# Autodesk Inventor assembly: Box_Tray_Assembly
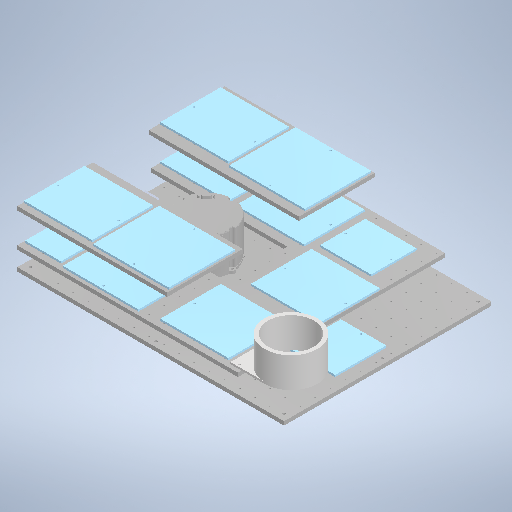
[picture p0: Inventor's stored thumbnail of the model, 512x512]
Saved by Autodesk Inventor 2025.3 (Build 293356000, 356)
## iProperties
Created: 2026-02-04
Part Number: Box_Tray_Assembly
Document SubType Name: Assembly
Designer: m263126
Author: m263126
## Documents named in this file (12)
- C:\Users\m263126\Documents\EW401 Capstone\CAD Files\Box_Tray_Assembly.iam
- C:\Users\m263126\Documents\EW401 Capstone\CAD Files\Box_Body.ipt
- C:\Users\m263126\Documents\EW401 Capstone\CAD Files\box tray_base.ipt
- C:\Users\m263126\Documents\EW401 Capstone\CAD Files\box tray_middle.ipt
- C:\Users\m263126\Documents\EW401 Capstone\CAD Files\box tray_top.ipt
- C:\Users\m263126\Documents\EW401 Capstone\CAD Files\Sensors\TAC-450\TAC-450 IMU.iam
- C:\Users\m263126\Documents\EW401 Capstone\CAD Files\Sensors\VN\vn100_rugged v2.iam
- C:\Users\m263126\Documents\EW401 Capstone\CAD Files\Brackets\4x2_bracket.ipt
- C:\Users\m263126\Documents\EW401 Capstone\CAD Files\Brackets\5x4_bracket.ipt
- C:\Users\m263126\Documents\EW401 Capstone\CAD Files\Brackets\4x4_bracket.ipt
- C:\Users\m263126\Documents\EW401 Capstone\CAD Files\Brackets\3x3_bracket.ipt
- C:\Users\m263126\Documents\EW401 Capstone\CAD Files\Brackets\Battery_holder2.ipt
## Components (19 placed, 11 different names)
1. Box_Body:1 — Mate:3, Mate:4
2. box tray_base:1 — Flush:1, Flush:2, Mate:1, Mate:3, Mate:4, Mate:5, Mate:6, Mate:7, Mate:8, Mate:9, Mate:41, Mate:42, Mate:43
3. box tray_middle:1 — Flush:1, Flush:2, Mate:1, Flush:3, Flush:4, Mate:2, Mate:25, Mate:26, Mate:27, Mate:28, Mate:29, Mate:30, Mate:31, Mate:33, Mate:34, Mate:37, Mate:38, Mate:39, Mate:40, Mate:44, Mate:45, Mate:46, Mate:47, Mate:48, Mate:49
4. box tray_top:1 — Flush:3, Flush:4, Mate:2, Mate:50, Mate:51, Mate:52, Mate:53, Mate:54, Mate:55, Mate:56, Mate:57, Mate:58, Mate:59, Mate:60, Mate:61
5. TAC-450 IMU:1 [sub-assembly] — Mate:5, Mate:6, Mate:7
6. vn100_rugged v2:1 [sub-assembly] — Mate:8, Mate:9
7. 4x4_bracket:2 — Mate:25, Mate:29, Mate:33
8. 4x4_bracket:3 — Mate:26, Mate:30, Mate:34
9. 4x4_bracket:4 — Mate:27
10. 4x4_bracket:5 — Mate:28, Mate:31, Mate:37
11. 5x4_bracket:1 — Mate:38, Mate:39, Mate:40
12. 5x4_bracket:2 — Mate:56, Mate:57, Mate:58
13. 5x4_bracket:3 — Mate:53, Mate:54, Mate:55
14. 3x3_bracket:1 — Mate:41, Mate:42, Mate:43
15. 3x3_bracket:2 — Mate:44, Mate:45, Mate:46
16. 4x2_bracket:1 — Mate:47, Mate:48, Mate:49
17. 4x4_bracket:6 — Mate:50, Mate:51, Mate:52
18. 4x4_bracket:7 — Mate:59, Mate:60, Mate:61
19. Battery_holder2:1
## Relationships (47: Mate 43, Flush 4)
- Flush:1: box tray_base:1 ↔ box tray_middle:1
- Flush:2: box tray_base:1 ↔ box tray_middle:1
- Mate:1 (25.4 mm): box tray_base:1 ↔ box tray_middle:1
- Flush:3: box tray_middle:1 ↔ box tray_top:1
- Flush:4: box tray_middle:1 ↔ box tray_top:1
- Mate:2 (50.8 mm): box tray_middle:1 ↔ box tray_top:1
- Mate:3: Box_Body:1 ↔ box tray_base:1
- Mate:4: Box_Body:1 ↔ box tray_base:1
- Mate:5: box tray_base:1 ↔ TAC-450 IMU:1
- Mate:6: box tray_base:1 ↔ TAC-450 IMU:1
- Mate:7: box tray_base:1 ↔ TAC-450 IMU:1
- Mate:8: box tray_base:1 ↔ vn100_rugged v2:1
- Mate:9: box tray_base:1 ↔ vn100_rugged v2:1
- Mate:25: box tray_middle:1 ↔ 4x4_bracket:2
- Mate:26: box tray_middle:1 ↔ 4x4_bracket:3
- Mate:27: box tray_middle:1 ↔ 4x4_bracket:4
- Mate:28: box tray_middle:1 ↔ 4x4_bracket:5
- Mate:29: box tray_middle:1 ↔ 4x4_bracket:2
- Mate:30: box tray_middle:1 ↔ 4x4_bracket:3
- Mate:31: box tray_middle:1 ↔ 4x4_bracket:5
- Mate:33: box tray_middle:1 ↔ 4x4_bracket:2
- Mate:34: box tray_middle:1 ↔ 4x4_bracket:3
- Mate:37: box tray_middle:1 ↔ 4x4_bracket:5
- Mate:38: box tray_middle:1 ↔ 5x4_bracket:1
- Mate:39: box tray_middle:1 ↔ 5x4_bracket:1
- Mate:40: box tray_middle:1 ↔ 5x4_bracket:1
- Mate:41: box tray_base:1 ↔ 3x3_bracket:1
- Mate:42: box tray_base:1 ↔ 3x3_bracket:1
- Mate:43: box tray_base:1 ↔ 3x3_bracket:1
- Mate:44: box tray_middle:1 ↔ 3x3_bracket:2
- Mate:45: box tray_middle:1 ↔ 3x3_bracket:2
- Mate:46: box tray_middle:1 ↔ 3x3_bracket:2
- Mate:47: box tray_middle:1 ↔ 4x2_bracket:1
- Mate:48: box tray_middle:1 ↔ 4x2_bracket:1
- Mate:49: box tray_middle:1 ↔ 4x2_bracket:1
- Mate:50: box tray_top:1 ↔ 4x4_bracket:6
- Mate:51: box tray_top:1 ↔ 4x4_bracket:6
- Mate:52: box tray_top:1 ↔ 4x4_bracket:6
- Mate:53: box tray_top:1 ↔ 5x4_bracket:3
- Mate:54: box tray_top:1 ↔ 5x4_bracket:3
- Mate:55: box tray_top:1 ↔ 5x4_bracket:3
- Mate:56: box tray_top:1 ↔ 5x4_bracket:2
- Mate:57: box tray_top:1 ↔ 5x4_bracket:2
- Mate:58: box tray_top:1 ↔ 5x4_bracket:2
- Mate:59: box tray_top:1 ↔ 4x4_bracket:7
- Mate:60: box tray_top:1 ↔ 4x4_bracket:7
- Mate:61: box tray_top:1 ↔ 4x4_bracket:7
